# Autodesk Inventor assembly: CoaxialSPM
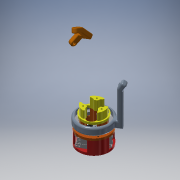
[picture p0: Inventor's stored thumbnail of the model, 180x180]
Saved by Autodesk Inventor 2019 (Build 230136000, 136)
## iProperties
Created: 2022-08-24
Part Number: CoaxialSPM
Document SubType Name: Assembly
Designer: zreik
Author: zreik
## Documents named in this file (12)
- D:\Documents\HIAST\4th year\4th Year Project\Design\Current\CoaxialSPM.iam
- D:\Documents\HIAST\4th year\4th Year Project\Design\Current\Base.ipt
- D:\Documents\HIAST\4th year\4th Year Project\Design\Current\XL-320.ipt
- D:\Documents\HIAST\4th year\4th Year Project\Design\Current\LayerBase1.ipt
- D:\Documents\HIAST\4th year\4th Year Project\Design\Current\LayerBase2.ipt
- D:\Documents\HIAST\4th year\4th Year Project\Design\Current\Layer1Gear.ipt
- D:\Documents\HIAST\4th year\4th Year Project\Design\Current\Layer2Gear.ipt
- D:\Documents\HIAST\4th year\4th Year Project\Design\Current\Layer3Gear.ipt
- D:\Documents\HIAST\4th year\4th Year Project\Design\Current\TopPlatform.ipt
- D:\Documents\HIAST\4th year\4th Year Project\Design\Current\Link.ipt
- D:\Documents\HIAST\4th year\4th Year Project\Design\Current\Motor1Gear.ipt
- D:\Documents\HIAST\4th year\4th Year Project\Design\Current\Bearing.ipt
## Components (14 placed, 11 different names)
1. Base:1 — Mate:1, Flush:1, Flush:2, Mate:12
2. LayerBase1:1 — Flush:2, Flush:3, Mate:11, Mate:12, Mate:13, Mate:14, Flush:4, Mate:17, Mate:38, Mate:39
3. LayerBase2:1 — Flush:3, Mate:10, Mate:13, Mate:14, Mate:15, Mate:16, Mate:18, Mate:19
4. LayerBase2:2 — Mate:10, Mate:15, Mate:16, Mate:20, Mate:21, Angle:2
5. Layer1Gear:1 — Flush:4, Mate:17, Mate:27
6. Layer2Gear:1 — Mate:18, Mate:19, Mate:25
7. Layer3Gear:1 — Mate:20, Mate:21, Mate:26
8. TopPlatform:1 — Mate:22, Mate:23, Mate:24, Angle:2, Mate:33
9. Link:1 — Mate:33
10. Motor1Gear:1 — Mate:34, Mate:35, Mate:36, Mate:37
11. Bearing:1 — Mate:38, Mate:39
12. XL-320:1 — Mate:1, Angle:1, Flush:1, Mate:2
13. XL-320:2 — Mate:34, Mate:35, Mate:36, Mate:37
14. XL-320:3
## Component patterns: (3 elements, first: XL-320:1)
## Relationships (38: Mate 32, Flush 4, Angle 2)
- Mate:1 (15 mm): Base:1 ↔ XL-320:1
- Angle:1 (0 deg): XL-320:1
- Flush:1 (-5 mm): Base:1 ↔ XL-320:1
- Mate:2: XL-320:1
- Flush:2: Base:1 ↔ LayerBase1:1
- Flush:3: LayerBase1:1 ↔ LayerBase2:1
- Mate:10: LayerBase2:1 ↔ LayerBase2:2
- Mate:11: LayerBase1:1
- Mate:12: Base:1 ↔ LayerBase1:1
- Mate:13: LayerBase1:1 ↔ LayerBase2:1
- Mate:14: LayerBase1:1 ↔ LayerBase2:1
- Mate:15: LayerBase2:1 ↔ LayerBase2:2
- Mate:16: LayerBase2:1 ↔ LayerBase2:2
- Flush:4: LayerBase1:1 ↔ Layer1Gear:1
- Mate:17: LayerBase1:1 ↔ Layer1Gear:1
- Mate:18: LayerBase2:1 ↔ Layer2Gear:1
- Mate:19: LayerBase2:1 ↔ Layer2Gear:1
- Mate:20: LayerBase2:2 ↔ Layer3Gear:1
- Mate:21: LayerBase2:2 ↔ Layer3Gear:1
- Mate:22: TopPlatform:1
- Mate:23: TopPlatform:1
- Mate:24: TopPlatform:1
- Mate:25: Layer2Gear:1
- Mate:26: Layer3Gear:1
- Mate:27: Layer1Gear:1
- Mate:28
- Mate:29
- Mate:30
- Mate:31
- Mate:32
- Angle:2 (0 deg): LayerBase2:2 ↔ TopPlatform:1
- Mate:33: TopPlatform:1 ↔ Link:1
- Mate:34: Motor1Gear:1 ↔ XL-320:2
- Mate:35: Motor1Gear:1 ↔ XL-320:2
- Mate:36: Motor1Gear:1 ↔ XL-320:2
- Mate:37: Motor1Gear:1 ↔ XL-320:2
- Mate:38: LayerBase1:1 ↔ Bearing:1
- Mate:39: LayerBase1:1 ↔ Bearing:1
